# Autodesk Inventor assembly: Kinematic-Mount Front [a]
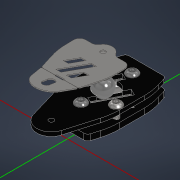
[picture p0: Inventor's stored thumbnail of the model, 180x180]
Saved by Autodesk Inventor 2022.2 (Build 262287010, 287A)
## iProperties
Created: 2022-03-13
Part Number: Kinematic-Mount Front [a]
Document SubType Name: Assembly
Designer: sleib
Author: sleib
## Documents named in this file (9)
- C:\Users\sleib\Projekte\Voron-2\CAD\Inventor\Kinematic-Mount Front [A].iam
- C:\Users\sleib\Projekte\Voron-2\CAD\Inventor\Kinematic-Bed Front-Support Bottom.ipt
- C:\Users\sleib\Projekte\Voron-2\CAD\Inventor\Pin 5x15.ipt
- C:\Users\sleib\Projekte\Voron-2\CAD\Inventor\Kinematic-Bed Front-Support Top.ipt
- C:\Users\sleib\Projekte\Voron-2\CAD\Inventor\M3x8 BHCS.ipt
- C:\Users\sleib\Projekte\Voron-2\CAD\Inventor\M3x12 BHCS.ipt
- C:\Users\sleib\Projekte\Voron-2\CAD\Inventor\M3 Threaded Ball.ipt
- C:\Users\sleib\Projekte\Voron-2\CAD\Inventor\M3x10x6 Standoff.ipt
- C:\Users\sleib\Projekte\Voron-2\CAD\Inventor\Kinematic-Bed Leaf-Spring.ipt
## Components (11 placed, 8 different names)
1. Kinematic-Bed Front-Support Bottom:1 — Passend:1, Passend:2, Passend:3, Passend:4, Passend:5, Passend:6, Passend:7, Passend:8, Passend:9, Passend:10, Passend:14, Passend:16, Passend:18, Passend:20
2. Kinematic-Bed Front-Support Top:1 — Passend:11, Passend:12, Passend:13, Passend:15, Passend:17, Passend:19, Passend:21, Passend:22, Passend:23, Passend:24, Passend:29
3. Kinematic-Bed Leaf-Spring:1 — Passend:27, Passend:28, Passend:29
4. M3 Threaded Ball:1 — Tangential:1, Tangential:2, Passend:25, Passend:26
5. M3x10x6 Standoff:1 — Passend:25, Passend:26, Passend:27, Passend:28
6. Pin 5x15:1 — Passend:5, Passend:6, Passend:10, Passend:11, Tangential:2
7. Pin 5x15:2 — Passend:7, Passend:8, Passend:9, Passend:12, Tangential:1
8. M3x8 BHCS:1 — Passend:13, Passend:14, Passend:24
9. M3x8 BHCS:2 — Passend:15, Passend:16, Passend:22
10. M3x12 BHCS:1 — Passend:19, Passend:20, Passend:21
11. M3x12 BHCS:2 — Passend:17, Passend:18, Passend:23
## Relationships (31: Mate 29, Tangent 2)
- Passend:1 [Mate]: Kinematic-Bed Front-Support Bottom:1
- Passend:2 [Mate]: Kinematic-Bed Front-Support Bottom:1
- Passend:3 [Mate]: Kinematic-Bed Front-Support Bottom:1
- Passend:4 [Mate]: Kinematic-Bed Front-Support Bottom:1
- Passend:5 [Mate] (2.5 mm): Kinematic-Bed Front-Support Bottom:1 ↔ Pin 5x15:1
- Passend:6 [Mate] (2.5 mm): Kinematic-Bed Front-Support Bottom:1 ↔ Pin 5x15:1
- Passend:7 [Mate] (2.5 mm): Kinematic-Bed Front-Support Bottom:1 ↔ Pin 5x15:2
- Passend:8 [Mate] (2.5 mm): Kinematic-Bed Front-Support Bottom:1 ↔ Pin 5x15:2
- Passend:9 [Mate] (0.2 mm): Kinematic-Bed Front-Support Bottom:1 ↔ Pin 5x15:2
- Passend:10 [Mate] (0.2 mm): Kinematic-Bed Front-Support Bottom:1 ↔ Pin 5x15:1
- Passend:11 [Mate] (2.5 mm): Kinematic-Bed Front-Support Top:1 ↔ Pin 5x15:1
- Passend:12 [Mate] (2.5 mm): Kinematic-Bed Front-Support Top:1 ↔ Pin 5x15:2
- Passend:13 [Mate]: Kinematic-Bed Front-Support Top:1 ↔ M3x8 BHCS:1
- Passend:14 [Mate]: Kinematic-Bed Front-Support Bottom:1 ↔ M3x8 BHCS:1
- Passend:15 [Mate]: Kinematic-Bed Front-Support Top:1 ↔ M3x8 BHCS:2
- Passend:16 [Mate]: Kinematic-Bed Front-Support Bottom:1 ↔ M3x8 BHCS:2
- Passend:17 [Mate]: Kinematic-Bed Front-Support Top:1 ↔ M3x12 BHCS:2
- Passend:18 [Mate]: Kinematic-Bed Front-Support Bottom:1 ↔ M3x12 BHCS:2
- Passend:19 [Mate]: Kinematic-Bed Front-Support Top:1 ↔ M3x12 BHCS:1
- Passend:20 [Mate]: Kinematic-Bed Front-Support Bottom:1 ↔ M3x12 BHCS:1
- Passend:21 [Mate]: Kinematic-Bed Front-Support Top:1 ↔ M3x12 BHCS:1
- Passend:22 [Mate]: Kinematic-Bed Front-Support Top:1 ↔ M3x8 BHCS:2
- Passend:23 [Mate]: Kinematic-Bed Front-Support Top:1 ↔ M3x12 BHCS:2
- Passend:24 [Mate]: Kinematic-Bed Front-Support Top:1 ↔ M3x8 BHCS:1
- Tangential:1: M3 Threaded Ball:1 ↔ Pin 5x15:2
- Tangential:2: M3 Threaded Ball:1 ↔ Pin 5x15:1
- Passend:25 [Mate]: M3 Threaded Ball:1 ↔ M3x10x6 Standoff:1
- Passend:26 [Mate] (1 mm): M3 Threaded Ball:1 ↔ M3x10x6 Standoff:1
- Passend:27 [Mate]: Kinematic-Bed Leaf-Spring:1 ↔ M3x10x6 Standoff:1
- Passend:28 [Mate]: Kinematic-Bed Leaf-Spring:1 ↔ M3x10x6 Standoff:1
- Passend:29 [Mate]: Kinematic-Bed Front-Support Top:1 ↔ Kinematic-Bed Leaf-Spring:1
